# Autodesk Inventor assembly: robot
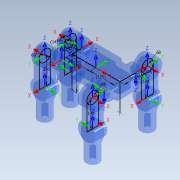
[picture p0: Inventor's stored thumbnail of the model, 180x180]
Saved by Autodesk Inventor 2020 (Build 240168000, 168)
## iProperties
Created: 2021-01-29
Part Number: robot
Document SubType Name: Assembly
Designer: DELL
Author: DELL
## Documents named in this file (7)
- F:\SoftRobot2.0\FlexipodFast\mesh\v7.0\robot.iam
- F:\SoftRobot2.0\FlexipodFast\mesh\v7.0\body.ipt
- F:\SoftRobot2.0\FlexipodFast\mesh\v7.0\hip.ipt
- F:\SoftRobot2.0\FlexipodFast\mesh\v7.0\thigh.ipt
- F:\SoftRobot2.0\FlexipodFast\mesh\v7.0\shank_2.ipt
- F:\SoftRobot2.0\FlexipodFast\mesh\v7.0\hip_back.ipt
- F:\SoftRobot2.0\FlexipodFast\mesh\v7.0\hip_back_mirror.ipt
## Components (13 placed, 6 different names)
1. body:1 — Flush:1, Flush:2, Flush:3, Mate:1, Mate:2, Mate:3, Mate:4, Angle:4, Angle:5, Angle:6, Angle:7, Angle:15, Angle:16, Angle:17, Mate:31, Mate:32, Mate:35, Mate:36, Angle:18
2. hip:1 — Mate:3, Mate:4, Mate:10, Mate:14, Angle:5
3. hip:2 — Mate:1, Mate:2, Mate:9, Flush:4, Angle:7
4. thigh:1 — Mate:9, Flush:4, Mate:30, Angle:17
5. thigh:2 — Mate:10, Mate:14, Mate:17, Angle:6
6. thigh:3 — Mate:16, Angle:16, Mate:33, Mate:34
7. thigh:4 — Mate:18, Angle:4, Angle:15, Flush:38, Mate:37, Angle:18
8. shank_2:1 — Mate:16
9. shank_2:2 — Mate:30
10. shank_2:3 — Mate:17
11. shank_2:4 — Mate:18
12. hip_back:1 — Mate:31, Mate:32, Mate:33, Mate:34
13. hip_back_mirror:1 — Mate:35, Mate:36, Flush:38, Mate:37
## Relationships (39: Mate 20, Angle 12, Flush 7)
- Flush:1: body:1
- Flush:2: body:1
- Flush:3: body:1
- Mate:1: body:1 ↔ hip:2
- Mate:2: body:1 ↔ hip:2
- Mate:3: body:1 ↔ hip:1
- Mate:4: body:1 ↔ hip:1
- Mate:9: hip:2 ↔ thigh:1
- Mate:10: hip:1 ↔ thigh:2
- Flush:4: hip:2 ↔ thigh:1
- Mate:14: hip:1 ↔ thigh:2
- Mate:16: thigh:3 ↔ shank_2:1
- Mate:17: thigh:2 ↔ shank_2:3
- Mate:18: thigh:4 ↔ shank_2:4
- [Mate]: thigh:4 ↔ shank_2:4
- [Flush]: thigh:3 ↔ shank_2:1
- [Flush]: thigh:2 ↔ shank_2:3
- [Mate]: thigh:1 ↔ shank_2:2
- Angle:4 (0 deg): body:1 ↔ thigh:4
- Angle:5 (0 deg): body:1 ↔ hip:1
- Angle:6 (0 deg): body:1 ↔ thigh:2
- Angle:7 (0 deg): body:1 ↔ hip:2
- [Angle] (0 deg): thigh:1 ↔ shank_2:2
- [Angle] (180 deg): thigh:2 ↔ shank_2:3
- [Angle] (0 deg): thigh:4 ↔ shank_2:4
- [Angle] (180 deg): thigh:3 ↔ shank_2:1
- Mate:30: thigh:1 ↔ shank_2:2
- Angle:15 (0 deg): body:1 ↔ thigh:4
- Angle:16 (0 deg): body:1 ↔ thigh:3
- Angle:17 (0 deg): body:1 ↔ thigh:1
- Mate:31: body:1 ↔ hip_back:1
- Mate:32: body:1 ↔ hip_back:1
- Mate:33: thigh:3 ↔ hip_back:1
- Mate:34: thigh:3 ↔ hip_back:1
- Mate:35: body:1 ↔ hip_back_mirror:1
- Mate:36: body:1 ↔ hip_back_mirror:1
- Flush:38: thigh:4 ↔ hip_back_mirror:1
- Mate:37: thigh:4 ↔ hip_back_mirror:1
- Angle:18 (0 deg): body:1 ↔ thigh:4
